# Autodesk Inventor assembly: relicGrabber
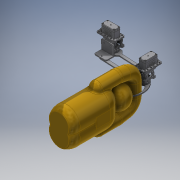
[picture p0: Inventor's stored thumbnail of the model, 180x180]
Saved by Autodesk Inventor 2018 (Build 220112000, 112)
## iProperties
Created: 2017-12-31
Part Number: relicGrabber
Document SubType Name: Assembly
Designer: mzhang
Author: mzhang
## Documents named in this file (12)
- C:\Users\mzhang\3D Objects\relicGrabber.iam
- C:\Users\mzhang\3D Objects\linkageMount.ipt
- C:\Users\mzhang\3D Objects\passiveLink.ipt
- C:\Users\mzhang\3D Objects\poweredArm.ipt
- C:\Users\mzhang\3D Objects\staticLink.ipt
- C:\Users\mzhang\Downloads\download (2)\637112\535118 assembly.ipt
- C:\Users\mzhang\Downloads\download (2)\637112\575112.ipt
- C:\Users\mzhang\Downloads\download (2)\637112\545420.ipt
- C:\Users\mzhang\Downloads\download (2)\637112\525123.ipt
- C:\Users\mzhang\Downloads\REV-41-1097.ipt
- C:\Users\mzhang\3D Objects\claw.ipt
- C:\Users\mzhang\Downloads\am-3570+Relic.ipt
## Components (18 placed, 11 different names)
1. linkageMount:1 — Mate:1, Mate:6, Mate:7, Mate:8, Mate:9
2. passiveLink:1 — Mate:1, Mate:5, Mate:6, Mate:43
3. poweredArm:1 — Mate:4, Mate:17, Mate:18, Mate:19, Mate:20, Mate:44
4. staticLink:1 — Mate:4, Mate:5, Mate:28, Mate:29, Mate:30, Mate:43, Mate:44
5. 535118 assembly:1 — Mate:10, Mate:11, Mate:12, Mate:13, Mate:14, Mate:15, Mate:16
6. 545420:1 — Mate:7, Mate:8, Mate:9, Mate:10, Mate:11, Mate:12, Mate:32
7. 525123:1 — Mate:16, Mate:17, Mate:18, Mate:19, Mate:20
8. 545420:2 — Mate:13, Mate:14, Mate:15, Mate:31, Mate:33
9. 535118 assembly:2 — Mate:42
10. 545420:3 — Mate:28, Mate:29, Mate:30, Mate:35
11. 525123:2 — Mate:39, Mate:40, Mate:41, Mate:42
12. 545420:4 — Mate:34, Mate:36
13. 575112:1 — Mate:31, Mate:32, Mate:33, Mate:38
14. 575112:2 — Mate:34, Mate:35, Mate:36, Mate:37
15. REV-41-1097:1 — Mate:38
16. REV-41-1097:2 — Mate:37
17. claw:1 — Mate:39, Mate:40, Mate:41
18. am-3570+Relic:1
## Relationships (42: Mate 42)
- Mate:1: linkageMount:1 ↔ passiveLink:1
- Mate:4: poweredArm:1 ↔ staticLink:1
- Mate:5: passiveLink:1 ↔ staticLink:1
- Mate:6: linkageMount:1 ↔ passiveLink:1
- Mate:7: linkageMount:1 ↔ 545420:1
- Mate:8: linkageMount:1 ↔ 545420:1
- Mate:9: linkageMount:1 ↔ 545420:1
- Mate:10: 535118 assembly:1 ↔ 545420:1
- Mate:11: 535118 assembly:1 ↔ 545420:1
- Mate:12: 535118 assembly:1 ↔ 545420:1
- Mate:13: 535118 assembly:1 ↔ 545420:2
- Mate:14: 535118 assembly:1 ↔ 545420:2
- Mate:15: 535118 assembly:1 ↔ 545420:2
- Mate:16: 535118 assembly:1 ↔ 525123:1
- Mate:17: poweredArm:1 ↔ 525123:1
- Mate:18: poweredArm:1 ↔ 525123:1
- Mate:19: poweredArm:1 ↔ 525123:1
- Mate:20: poweredArm:1 ↔ 525123:1
- [Mate]: 535118 assembly:2 ↔ 545420:3
- [Mate]: 535118 assembly:2 ↔ 545420:3
- [Mate]: 535118 assembly:2 ↔ 545420:3
- [Mate]: 535118 assembly:2 ↔ 545420:4
- [Mate]: 535118 assembly:2 ↔ 545420:4
- [Mate]: 535118 assembly:2 ↔ 545420:4
- [Mate]: 535118 assembly:2 ↔ 525123:2
- Mate:28: staticLink:1 ↔ 545420:3
- Mate:29: staticLink:1 ↔ 545420:3
- Mate:30: staticLink:1 ↔ 545420:3
- Mate:31: 545420:2 ↔ 575112:1
- Mate:32: 545420:1 ↔ 575112:1
- Mate:33: 545420:2 ↔ 575112:1
- Mate:34: 545420:4 ↔ 575112:2
- Mate:35: 545420:3 ↔ 575112:2
- Mate:36: 545420:4 ↔ 575112:2
- Mate:37: 575112:2 ↔ REV-41-1097:2
- Mate:38: 575112:1 ↔ REV-41-1097:1
- Mate:39: 525123:2 ↔ claw:1
- Mate:40: 525123:2 ↔ claw:1
- Mate:41: 525123:2 ↔ claw:1
- Mate:42 (6 mm): 535118 assembly:2 ↔ 525123:2
- Mate:43: passiveLink:1 ↔ staticLink:1
- Mate:44: poweredArm:1 ↔ staticLink:1
## Named parameters: d21_d10 = 0 mm, d22_d11 = 0 mm, d23_d12 = 0 mm, d24_d13 = 0 mm, d25_d14 = 0 mm, d26_d15 = 0 mm, d27_d16 = 0 mm
